# Autodesk Inventor assembly: stackedSpool
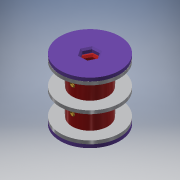
[picture p0: Inventor's stored thumbnail of the model, 180x180]
Saved by Autodesk Inventor 2019.3 (Build 233278000, 278)
## iProperties
Created: 2019-03-05
Part Number: stackedSpool
Document SubType Name: Assembly
Designer: steele
Author: steele
## Documents named in this file (5)
- C:\git\CAD-Development\robSteele\RevRoboticsExtrusionAttachements\stackedSpool.iam
- C:\git\CAD-Development\robSteele\RevRoboticsExtrusionAttachements\spacerForEnd.ipt
- C:\git\CAD-Development\robSteele\RevRoboticsExtrusionAttachements\washer2_5x1_0.ipt
- c:\git\CAD-MfgResources\McMaster-Carr\BrassHeatSetInsertForPlastic\6-32 0_281 94459A290_BRASS HEAT-SET INSERT FOR PLASTIC.ipt
- C:\git\CAD-Development\robSteele\RevRoboticsExtrusionAttachements\spoolV04.ipt
## Components (9 placed, 4 different names)
1. spacerForEnd:1 — Insert:1
2. washer2_5x1_0:1 — Insert:1, Insert:2
3. spoolV04:1 — Insert:2, Insert:3, Insert:8
4. washer2_5x1_0:2 — Insert:3, Insert:4
5. spoolV04:2 — Insert:4, Insert:5, Insert:7
6. washer2_5x1_0:3 — Insert:5, Insert:6
7. spacerForEnd:2 — Insert:6
8. 6-32 0_281 94459A290_BRASS HEAT-SET INSERT FOR PLASTIC:1 — Insert:7
9. 6-32 0_281 94459A290_BRASS HEAT-SET INSERT FOR PLASTIC:2 — Insert:8
## Relationships (8: Insert 8)
- Insert:1: spacerForEnd:1 ↔ washer2_5x1_0:1
- Insert:2: washer2_5x1_0:1 ↔ spoolV04:1
- Insert:3: spoolV04:1 ↔ washer2_5x1_0:2
- Insert:4: washer2_5x1_0:2 ↔ spoolV04:2
- Insert:5: spoolV04:2 ↔ washer2_5x1_0:3
- Insert:6 (-1.016 mm): washer2_5x1_0:3 ↔ spacerForEnd:2
- Insert:7: spoolV04:2 ↔ 6-32 0_281 94459A290_BRASS HEAT-SET INSERT FOR PLASTIC:1
- Insert:8: spoolV04:1 ↔ 6-32 0_281 94459A290_BRASS HEAT-SET INSERT FOR PLASTIC:2
